# Autodesk Inventor assembly: MX-106T_with_Horn_Schwung
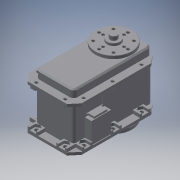
[picture p0: Inventor's stored thumbnail of the model, 180x180]
Saved by Autodesk Inventor 2016 (Build 200138000, 138)
## iProperties
Created: 2015-05-09
Part Number: MX-106T_with_Horn_Schwung
Document SubType Name: Assembly
Designer: bitbots
Mass: 86.5151 g
Surface Area: 177.097 cm^2
Volume: 86.5151 cm^3
Density: 1 g/cm^3
Author: bitbots
## Documents named in this file (4)
- Z:\nimbro_cad\NICU Assembly(ADI)_new\motors_new\Mx106\MX-106T_with_Horn_Schwung.iam
- Z:\nimbro_cad\NICU Assembly(ADI)_new\motors_new\Mx106\MX-106T.ipt
- Z:\nimbro_cad\NICU Assembly(ADI)_new\motors_new\HN05-N101_(mx64)\HN05-N101.ipt
- Z:\nimbro_cad\NICU Assembly(ADI)_new\motors_new\HN05-i1_(mx64_bearing)\Imported Components\HN05-i1\HN05-i1.ipt
## Components (3 placed, 3 different names)
1. MX-106T:1 — Rotational:1, Rotational:2
2. HN05-N101:1 — Rotational:1
3. HN05-i1:1 — Rotational:2
## Relationships (2: RevoluteJoint 2)
- Rotational:1 [RevoluteJoint] (-7 mm): MX-106T:1 ↔ HN05-N101:1
- Rotational:2 [RevoluteJoint]: MX-106T:1 ↔ HN05-i1:1
